# Autodesk Inventor assembly: Plastic Clamping Bearing Block Pair.ipt
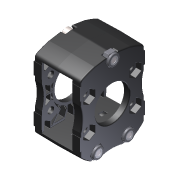
[picture p0: Inventor's stored thumbnail of the model, 180x180]
Saved by Autodesk Inventor 2015 (Build 190159000, 159)
## iProperties
Created: 2014-12-18
Part Number: Plastic Clamping Bearing Block Pair.ipt
Document SubType Name: Assembly
Designer: Nemo
Author: Nemo
## Documents named in this file (4)
- H:\Nemo\Documents\Robotics\CAD Files\COTS Parts\VersaFrame\Plastic Clamping Bearing Block Pair.ipt.iam
- H:\Nemo\Documents\Robotics\CAD Files\COTS Parts\VersaFrame\Plastic Clamping Bearing Block.ipt
- H:\Nemo\Documents\Robotics\CAD Files\COTS Parts\Fasteners\10-32\10-32 locknut.ipt
- H:\Nemo\Documents\Robotics\CAD Files\COTS Parts\Fasteners\10-32\10-32 SHCS x1375.ipt
## Components (8 placed, 3 different names)
1. Plastic Clamping Bearing Block:1 — Mate:1, Flush:2, Mate:6, Insert:4, Insert:5, Insert:6, Flush:3
2. Plastic Clamping Bearing Block:2 — Flush:1, Mate:4, Mate:6, Insert:1, Insert:2, Insert:3
3. 10-32 locknut:1 — Insert:1
4. 10-32 locknut:2 — Insert:2
5. 10-32 locknut:3 — Insert:3
6. 10-32 SHCS x1375:1 — Insert:4
7. 10-32 SHCS x1375:2 — Insert:5
8. 10-32 SHCS x1375:3 — Insert:6
## Relationships (12: Insert 6, Mate 3, Flush 3)
- Mate:1: Plastic Clamping Bearing Block:1
- Flush:1: Plastic Clamping Bearing Block:2
- Flush:2: Plastic Clamping Bearing Block:1
- Mate:4: Plastic Clamping Bearing Block:2
- Mate:6: Plastic Clamping Bearing Block:1 ↔ Plastic Clamping Bearing Block:2
- Insert:1: Plastic Clamping Bearing Block:2 ↔ 10-32 locknut:1
- Insert:2: Plastic Clamping Bearing Block:2 ↔ 10-32 locknut:2
- Insert:3: Plastic Clamping Bearing Block:2 ↔ 10-32 locknut:3
- Insert:4: Plastic Clamping Bearing Block:1 ↔ 10-32 SHCS x1375:1
- Insert:5: Plastic Clamping Bearing Block:1 ↔ 10-32 SHCS x1375:2
- Insert:6: Plastic Clamping Bearing Block:1 ↔ 10-32 SHCS x1375:3
- Flush:3: Plastic Clamping Bearing Block:1
